# Autodesk Inventor assembly: Intake Full Assembly
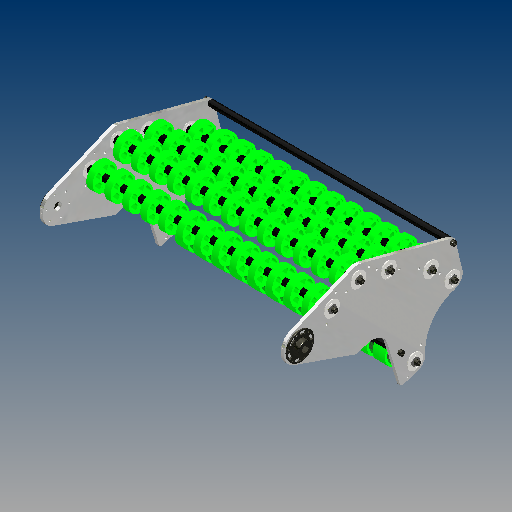
[picture p0: Inventor's stored thumbnail of the model, 512x512]
Saved by Autodesk Inventor 2024.3 (Build 283343000, 343)
## iProperties
Created: 2024-07-29
Part Number: Intake Full Assembly
Document SubType Name: Assembly
Designer: Kenji
Author: Kenji
## Documents named in this file (10)
- C:\Users\Kenji\Documents\GitHub\1622-2024-Summer-CAD-A-Thon\Intake\Intake Full Assembly.iam
- C:\Users\Kenji\Documents\GitHub\1622-2024-Summer-CAD-A-Thon\Intake\Intake Roller Plate.ipt
- C:\Users\Kenji\Documents\GitHub\1622-2024-Summer-CAD-A-Thon\COTS Library\Motion\Bearings\COTS_WCP-0783_1.125ODHexBearing.ipt
- C:\Users\Kenji\Documents\GitHub\1622-2024-Summer-CAD-A-Thon\Intake\Intake HexShaft 1.ipt
- C:\Users\Kenji\Documents\GitHub\1622-2024-Summer-CAD-A-Thon\COTS Library\Motion\Wheels\Compliant Wheels\2in compliant wheels\0.500in hex bore\COTS_am-3462_2indiameter_0.500inhexbore_durometer35A_CompliantWheel.ipt
- C:\Users\Kenji\Documents\GitHub\1622-2024-Summer-CAD-A-Thon\COTS Library\Motion\Wheels\Stealth Wheels\COTS_am-3155 2IN 500Hex Stealth Wheel.iam
- C:\Users\Kenji\Documents\GitHub\1622-2024-Summer-CAD-A-Thon\COTS Library\Structural Adapter\VersaHubs\COTS_217-2592_VersaHub.ipt
- C:\Users\Kenji\Documents\GitHub\1622-2024-Summer-CAD-A-Thon\Intake\Intake BeaterBar.ipt
- C:\Users\Kenji\Documents\GitHub\1622-2024-Summer-CAD-A-Thon\COTS Library\Fasteners\Bolts\Socket-Head\0.25-20\COTS_91251A539_Black-Oxide Alloy Steel Socket Head Screw (1).ipt
- C:\Users\Kenji\Documents\GitHub\1622-2024-Summer-CAD-A-Thon\COTS Library\Fasteners\Washers\COTS_90107A029_316 Stainless Steel Washer.ipt
## Components (129 placed, 9 different names)
1. Intake Roller Plate:1 — Mate:225, Mate:226, Mate:227, Mate:228, Mate:234, Mate:235, Mate:240, Mate:241, Mate:242, Mate:243, Mate:244, Mate:245, Mate:246, Mate:254, Mate:255, Mate:256, Mate:257
2. Intake Roller Plate:2 — Mate:226, Mate:227, Mate:229, Mate:230, Mate:231, Mate:232, Mate:236, Mate:237, Mate:238, Mate:239, Mate:247, Mate:248, Mate:249, Mate:250, Mate:252, Mate:258, Mate:259, Mate:260, Mate:261
3. COTS_WCP-0783_1.125ODHexBearing:1 — Mate:25, Mate:32, Flush:11, Mate:229, Mate:230
4. COTS_WCP-0783_1.125ODHexBearing:2 — Mate:26, Mate:27, Flush:1
5. COTS_WCP-0783_1.125ODHexBearing:3 — Mate:31, Flush:9, Mate:236, Mate:237
6. COTS_WCP-0783_1.125ODHexBearing:4 — Flush:8, Mate:231, Mate:232, Mate:233
7. COTS_WCP-0783_1.125ODHexBearing:5 — Flush:4, Mate:238, Mate:239
8. COTS_WCP-0783_1.125ODHexBearing:6 — Flush:6, Mate:261
9. COTS_WCP-0783_1.125ODHexBearing:7 — Flush:10, Mate:115, Mate:135
10. COTS_WCP-0783_1.125ODHexBearing:8 — Mate:30, Flush:7, Mate:130
11. COTS_WCP-0783_1.125ODHexBearing:9 — Mate:29, Flush:5, Mate:134, Mate:234, Mate:235
12. COTS_WCP-0783_1.125ODHexBearing:10 — Mate:25, Flush:12, Mate:136, Mate:225, Mate:228
13. COTS_WCP-0783_1.125ODHexBearing:11 — Mate:26, Flush:2, Mate:132, Mate:144, Mate:241, Mate:242
14. COTS_WCP-0783_1.125ODHexBearing:12 — Mate:28, Flush:3, Mate:33, Mate:133, Mate:240
15. Intake HexShaft 1:1 — Mate:31, Flush:9, Flush:10, Mate:85, Mate:115, Mate:177, Mate:178, Mate:206, Mate:223
16. Intake HexShaft 1:2 — Mate:32, Flush:11, Flush:12, Mate:98, Mate:183, Mate:184, Mate:209, Mate:220
17. Intake HexShaft 1:3 — Mate:30, Flush:7, Flush:8, Mate:72, Mate:181, Mate:182, Mate:208, Mate:221
18. Intake HexShaft 1:4 — Mate:29, Flush:5, Flush:6, Mate:59, Mate:179, Mate:180, Mate:207, Mate:222
19. Intake HexShaft 1:5 — Mate:28, Flush:3, Flush:4, Mate:175, Mate:176, Mate:205, Mate:224
20. Intake HexShaft 1:6 — Mate:27, Flush:1, Flush:2, Mate:173, Mate:174, Mate:201, Mate:202, Mate:203
21. COTS_217-2592_VersaHub:2 — Mate:255, Mate:256, Mate:257
22. COTS_217-2592_VersaHub:3 — Mate:258, Mate:259, Mate:260
23. Intake BeaterBar:1 — Mate:251, Mate:252
24. Intake BeaterBar:2 — Mate:253, Mate:254
25. COTS_91251A539_Black-Oxide Alloy Steel Socket Head Screw (1):1 — Mate:212, Mate:213
26. COTS_91251A539_Black-Oxide Alloy Steel Socket Head Screw (1):2 — Mate:243, Mate:244, Mate:253
27. COTS_91251A539_Black-Oxide Alloy Steel Socket Head Screw (1):3 — Mate:214, Mate:215
28. COTS_91251A539_Black-Oxide Alloy Steel Socket Head Screw (1):4 — Mate:201, Mate:204
29. COTS_91251A539_Black-Oxide Alloy Steel Socket Head Screw (1):5 — Mate:195, Mate:196
30. COTS_91251A539_Black-Oxide Alloy Steel Socket Head Screw (1):6 — Mate:210, Mate:211
31. COTS_91251A539_Black-Oxide Alloy Steel Socket Head Screw (1):7 — Mate:189, Mate:190
32. COTS_91251A539_Black-Oxide Alloy Steel Socket Head Screw (1):8 — Mate:193, Mate:194
33. COTS_91251A539_Black-Oxide Alloy Steel Socket Head Screw (1):9 — Mate:249, Mate:250, Mate:251
34. COTS_91251A539_Black-Oxide Alloy Steel Socket Head Screw (1):10 — Mate:247, Mate:248
35. COTS_91251A539_Black-Oxide Alloy Steel Socket Head Screw (1):11 — Mate:216, Mate:217
36. COTS_91251A539_Black-Oxide Alloy Steel Socket Head Screw (1):12 — Mate:218, Mate:219
37. COTS_91251A539_Black-Oxide Alloy Steel Socket Head Screw (1):13 — Mate:245, Mate:246
38. COTS_91251A539_Black-Oxide Alloy Steel Socket Head Screw (1):14 — Mate:191, Mate:192
39. COTS_91251A539_Black-Oxide Alloy Steel Socket Head Screw (1):15 — Mate:187, Mate:188, Mate:233
40. COTS_91251A539_Black-Oxide Alloy Steel Socket Head Screw (1):16 — Mate:185, Mate:186
41. COTS_90107A029_316 Stainless Steel Washer:1 — Mate:206, Mate:212, Mate:213, Mate:223
42. COTS_90107A029_316 Stainless Steel Washer:2 — Mate:207, Mate:214, Mate:215, Mate:222
43. COTS_90107A029_316 Stainless Steel Washer:3 — Mate:175, Mate:176, Mate:193, Mate:194
44. COTS_90107A029_316 Stainless Steel Washer:4 — Mate:208, Mate:216, Mate:217, Mate:221
45. COTS_90107A029_316 Stainless Steel Washer:5 — Mate:181, Mate:182, Mate:187, Mate:188
46. COTS_90107A029_316 Stainless Steel Washer:6 — Mate:205, Mate:210, Mate:211, Mate:224
47. COTS_90107A029_316 Stainless Steel Washer:7 — Mate:202, Mate:203, Mate:204
48. COTS_90107A029_316 Stainless Steel Washer:8 — Mate:183, Mate:184, Mate:185, Mate:186
49. COTS_90107A029_316 Stainless Steel Washer:9 — Mate:209, Mate:218, Mate:219, Mate:220
50. COTS_90107A029_316 Stainless Steel Washer:10 — Mate:179, Mate:180, Mate:189, Mate:190
51. COTS_90107A029_316 Stainless Steel Washer:11 — Mate:173, Mate:174, Mate:195, Mate:196
52. COTS_90107A029_316 Stainless Steel Washer:12 — Mate:177, Mate:178, Mate:191, Mate:192
53. COTS_am-3462_2indiameter_0.500inhexbore_durometer35A_CompliantWheel:40 — Mate:72, Mate:130
54. COTS_am-3462_2indiameter_0.500inhexbore_durometer35A_CompliantWheel:53 — Mate:85, Mate:135
55. COTS_am-3462_2indiameter_0.500inhexbore_durometer35A_CompliantWheel:25 — Mate:59, Mate:134
56. COTS_am-3462_2indiameter_0.500inhexbore_durometer35A_CompliantWheel:24 — Mate:33, Mate:133
57. COTS_am-3462_2indiameter_0.500inhexbore_durometer35A_CompliantWheel:66 — Mate:98, Mate:136
58. COTS_am-3462_2indiameter_0.500inhexbore_durometer35A_CompliantWheel:67
59. COTS_am-3462_2indiameter_0.500inhexbore_durometer35A_CompliantWheel:68
60. COTS_am-3462_2indiameter_0.500inhexbore_durometer35A_CompliantWheel:69
61. COTS_am-3462_2indiameter_0.500inhexbore_durometer35A_CompliantWheel:70
62. COTS_am-3462_2indiameter_0.500inhexbore_durometer35A_CompliantWheel:95
63. COTS_am-3462_2indiameter_0.500inhexbore_durometer35A_CompliantWheel:71
64. COTS_am-3462_2indiameter_0.500inhexbore_durometer35A_CompliantWheel:72
65. COTS_am-3462_2indiameter_0.500inhexbore_durometer35A_CompliantWheel:73
66. COTS_am-3462_2indiameter_0.500inhexbore_durometer35A_CompliantWheel:74
67. COTS_am-3462_2indiameter_0.500inhexbore_durometer35A_CompliantWheel:96
68. COTS_am-3462_2indiameter_0.500inhexbore_durometer35A_CompliantWheel:75
69. COTS_am-3462_2indiameter_0.500inhexbore_durometer35A_CompliantWheel:76
70. COTS_am-3462_2indiameter_0.500inhexbore_durometer35A_CompliantWheel:77
71. COTS_am-3462_2indiameter_0.500inhexbore_durometer35A_CompliantWheel:78
72. COTS_am-3462_2indiameter_0.500inhexbore_durometer35A_CompliantWheel:97
73. COTS_am-3462_2indiameter_0.500inhexbore_durometer35A_CompliantWheel:79
74. COTS_am-3462_2indiameter_0.500inhexbore_durometer35A_CompliantWheel:80
75. COTS_am-3462_2indiameter_0.500inhexbore_durometer35A_CompliantWheel:81
76. COTS_am-3462_2indiameter_0.500inhexbore_durometer35A_CompliantWheel:82
77. COTS_am-3462_2indiameter_0.500inhexbore_durometer35A_CompliantWheel:98
78. COTS_am-3462_2indiameter_0.500inhexbore_durometer35A_CompliantWheel:83
79. COTS_am-3462_2indiameter_0.500inhexbore_durometer35A_CompliantWheel:84
80. COTS_am-3462_2indiameter_0.500inhexbore_durometer35A_CompliantWheel:85
81. COTS_am-3462_2indiameter_0.500inhexbore_durometer35A_CompliantWheel:86
82. COTS_am-3462_2indiameter_0.500inhexbore_durometer35A_CompliantWheel:99
83. COTS_am-3462_2indiameter_0.500inhexbore_durometer35A_CompliantWheel:87
84. COTS_am-3462_2indiameter_0.500inhexbore_durometer35A_CompliantWheel:88
85. COTS_am-3462_2indiameter_0.500inhexbore_durometer35A_CompliantWheel:89
86. COTS_am-3462_2indiameter_0.500inhexbore_durometer35A_CompliantWheel:90
87. COTS_am-3462_2indiameter_0.500inhexbore_durometer35A_CompliantWheel:100
88. COTS_am-3462_2indiameter_0.500inhexbore_durometer35A_CompliantWheel:91
89. COTS_am-3462_2indiameter_0.500inhexbore_durometer35A_CompliantWheel:92
90. COTS_am-3462_2indiameter_0.500inhexbore_durometer35A_CompliantWheel:93
91. COTS_am-3462_2indiameter_0.500inhexbore_durometer35A_CompliantWheel:94
92. COTS_am-3462_2indiameter_0.500inhexbore_durometer35A_CompliantWheel:101
93. COTS_am-3462_2indiameter_0.500inhexbore_durometer35A_CompliantWheel:102
94. COTS_am-3462_2indiameter_0.500inhexbore_durometer35A_CompliantWheel:103
95. COTS_am-3462_2indiameter_0.500inhexbore_durometer35A_CompliantWheel:104
96. COTS_am-3462_2indiameter_0.500inhexbore_durometer35A_CompliantWheel:105
97. COTS_am-3462_2indiameter_0.500inhexbore_durometer35A_CompliantWheel:106
98. COTS_am-3462_2indiameter_0.500inhexbore_durometer35A_CompliantWheel:107
99. COTS_am-3462_2indiameter_0.500inhexbore_durometer35A_CompliantWheel:108
100. COTS_am-3462_2indiameter_0.500inhexbore_durometer35A_CompliantWheel:109
101. COTS_am-3462_2indiameter_0.500inhexbore_durometer35A_CompliantWheel:110
102. COTS_am-3462_2indiameter_0.500inhexbore_durometer35A_CompliantWheel:111
103. COTS_am-3462_2indiameter_0.500inhexbore_durometer35A_CompliantWheel:112
104. COTS_am-3462_2indiameter_0.500inhexbore_durometer35A_CompliantWheel:113
105. COTS_am-3462_2indiameter_0.500inhexbore_durometer35A_CompliantWheel:114
106. COTS_am-3462_2indiameter_0.500inhexbore_durometer35A_CompliantWheel:115
107. COTS_am-3462_2indiameter_0.500inhexbore_durometer35A_CompliantWheel:116
108. COTS_am-3462_2indiameter_0.500inhexbore_durometer35A_CompliantWheel:117
109. COTS_am-3462_2indiameter_0.500inhexbore_durometer35A_CompliantWheel:118
110. COTS_am-3462_2indiameter_0.500inhexbore_durometer35A_CompliantWheel:119
111. COTS_am-3462_2indiameter_0.500inhexbore_durometer35A_CompliantWheel:120
112. COTS_am-3462_2indiameter_0.500inhexbore_durometer35A_CompliantWheel:121
113. COTS_am-3462_2indiameter_0.500inhexbore_durometer35A_CompliantWheel:122
114. COTS_am-3462_2indiameter_0.500inhexbore_durometer35A_CompliantWheel:123
115. COTS_am-3462_2indiameter_0.500inhexbore_durometer35A_CompliantWheel:124
116. COTS_am-3462_2indiameter_0.500inhexbore_durometer35A_CompliantWheel:125
117. COTS_am-3462_2indiameter_0.500inhexbore_durometer35A_CompliantWheel:126
118. COTS_am-3155 2IN 500Hex Stealth Wheel:7 [sub-assembly] — Mate:132, Mate:144
119. COTS_am-3155 2IN 500Hex Stealth Wheel:8 [sub-assembly]
120. COTS_am-3155 2IN 500Hex Stealth Wheel:9 [sub-assembly]
121. COTS_am-3155 2IN 500Hex Stealth Wheel:10 [sub-assembly]
122. COTS_am-3155 2IN 500Hex Stealth Wheel:11 [sub-assembly]
123. COTS_am-3155 2IN 500Hex Stealth Wheel:12 [sub-assembly]
124. COTS_am-3155 2IN 500Hex Stealth Wheel:13 [sub-assembly]
125. COTS_am-3155 2IN 500Hex Stealth Wheel:14 [sub-assembly]
126. COTS_am-3155 2IN 500Hex Stealth Wheel:15 [sub-assembly]
127. COTS_am-3155 2IN 500Hex Stealth Wheel:16 [sub-assembly]
128. COTS_am-3155 2IN 500Hex Stealth Wheel:17 [sub-assembly]
129. COTS_am-3155 2IN 500Hex Stealth Wheel:18 [sub-assembly]
## Component patterns: (13 elements, first: COTS_am-3462_2indiameter_0.500inhexbore_durometer35A_CompliantWheel:40 + COTS_am-3462_2indiameter_0.500inhexbore_durometer35A_CompliantWheel:53 + COTS_am-3462_2indiameter_0.500inhexbore_durometer35A_CompliantWheel:25 + COTS_am-3462_2indiameter_0.500inhexbore_durometer35A_CompliantWheel:24 + COTS_am-3462_2indiameter_0.500inhexbore_durometer35A_CompliantWheel:66), (12 elements, first: COTS_am-3155 2IN 500Hex Stealth Wheel:7)
## Relationships (118: Mate 106, Flush 12)
- Mate:25: COTS_WCP-0783_1.125ODHexBearing:1 ↔ COTS_WCP-0783_1.125ODHexBearing:10
- Mate:26: COTS_WCP-0783_1.125ODHexBearing:2 ↔ COTS_WCP-0783_1.125ODHexBearing:11
- Mate:27: COTS_WCP-0783_1.125ODHexBearing:2 ↔ Intake HexShaft 1:6
- Flush:1: COTS_WCP-0783_1.125ODHexBearing:2 ↔ Intake HexShaft 1:6
- Flush:2: COTS_WCP-0783_1.125ODHexBearing:11 ↔ Intake HexShaft 1:6
- Mate:28: COTS_WCP-0783_1.125ODHexBearing:12 ↔ Intake HexShaft 1:5
- Flush:3: COTS_WCP-0783_1.125ODHexBearing:12 ↔ Intake HexShaft 1:5
- Flush:4: COTS_WCP-0783_1.125ODHexBearing:5 ↔ Intake HexShaft 1:5
- Mate:29: COTS_WCP-0783_1.125ODHexBearing:9 ↔ Intake HexShaft 1:4
- Flush:5: COTS_WCP-0783_1.125ODHexBearing:9 ↔ Intake HexShaft 1:4
- Flush:6: COTS_WCP-0783_1.125ODHexBearing:6 ↔ Intake HexShaft 1:4
- Mate:30: COTS_WCP-0783_1.125ODHexBearing:8 ↔ Intake HexShaft 1:3
- Flush:7: COTS_WCP-0783_1.125ODHexBearing:8 ↔ Intake HexShaft 1:3
- Flush:8: COTS_WCP-0783_1.125ODHexBearing:4 ↔ Intake HexShaft 1:3
- Mate:31: COTS_WCP-0783_1.125ODHexBearing:3 ↔ Intake HexShaft 1:1
- Flush:9: COTS_WCP-0783_1.125ODHexBearing:3 ↔ Intake HexShaft 1:1
- Flush:10: COTS_WCP-0783_1.125ODHexBearing:7 ↔ Intake HexShaft 1:1
- Mate:32: COTS_WCP-0783_1.125ODHexBearing:1 ↔ Intake HexShaft 1:2
- Flush:11: COTS_WCP-0783_1.125ODHexBearing:1 ↔ Intake HexShaft 1:2
- Flush:12: COTS_WCP-0783_1.125ODHexBearing:10 ↔ Intake HexShaft 1:2
- Mate:33: COTS_WCP-0783_1.125ODHexBearing:12 ↔ COTS_am-3462_2indiameter_0.500inhexbore_durometer35A_CompliantWheel:24
- Mate:59: Intake HexShaft 1:4 ↔ COTS_am-3462_2indiameter_0.500inhexbore_durometer35A_CompliantWheel:25
- Mate:72: Intake HexShaft 1:3 ↔ COTS_am-3462_2indiameter_0.500inhexbore_durometer35A_CompliantWheel:40
- Mate:85: Intake HexShaft 1:1 ↔ COTS_am-3462_2indiameter_0.500inhexbore_durometer35A_CompliantWheel:53
- Mate:98: Intake HexShaft 1:2 ↔ COTS_am-3462_2indiameter_0.500inhexbore_durometer35A_CompliantWheel:66
- Mate:115: COTS_WCP-0783_1.125ODHexBearing:7 ↔ Intake HexShaft 1:1
- Mate:130 (15.24 mm): COTS_WCP-0783_1.125ODHexBearing:8 ↔ COTS_am-3462_2indiameter_0.500inhexbore_durometer35A_CompliantWheel:40
- Mate:132 (27.94 mm): COTS_WCP-0783_1.125ODHexBearing:11 ↔ COTS_am-3155 2IN 500Hex Stealth Wheel:7
- Mate:133 (15.24 mm): COTS_WCP-0783_1.125ODHexBearing:12 ↔ COTS_am-3462_2indiameter_0.500inhexbore_durometer35A_CompliantWheel:24
- Mate:134 (15.24 mm): COTS_WCP-0783_1.125ODHexBearing:9 ↔ COTS_am-3462_2indiameter_0.500inhexbore_durometer35A_CompliantWheel:25
- Mate:135 (15.24 mm): COTS_WCP-0783_1.125ODHexBearing:7 ↔ COTS_am-3462_2indiameter_0.500inhexbore_durometer35A_CompliantWheel:53
- Mate:136 (15.24 mm): COTS_WCP-0783_1.125ODHexBearing:10 ↔ COTS_am-3462_2indiameter_0.500inhexbore_durometer35A_CompliantWheel:66
- Mate:144: COTS_WCP-0783_1.125ODHexBearing:11 ↔ COTS_am-3155 2IN 500Hex Stealth Wheel:7
- Mate:173: Intake HexShaft 1:6 ↔ COTS_90107A029_316 Stainless Steel Washer:11
- Mate:174: Intake HexShaft 1:6 ↔ COTS_90107A029_316 Stainless Steel Washer:11
- Mate:175: Intake HexShaft 1:5 ↔ COTS_90107A029_316 Stainless Steel Washer:3
- Mate:176: Intake HexShaft 1:5 ↔ COTS_90107A029_316 Stainless Steel Washer:3
- Mate:177: Intake HexShaft 1:1 ↔ COTS_90107A029_316 Stainless Steel Washer:12
- Mate:178: Intake HexShaft 1:1 ↔ COTS_90107A029_316 Stainless Steel Washer:12
- Mate:179: Intake HexShaft 1:4 ↔ COTS_90107A029_316 Stainless Steel Washer:10
- Mate:180: Intake HexShaft 1:4 ↔ COTS_90107A029_316 Stainless Steel Washer:10
- Mate:181: Intake HexShaft 1:3 ↔ COTS_90107A029_316 Stainless Steel Washer:5
- Mate:182: Intake HexShaft 1:3 ↔ COTS_90107A029_316 Stainless Steel Washer:5
- Mate:183: Intake HexShaft 1:2 ↔ COTS_90107A029_316 Stainless Steel Washer:8
- Mate:184: Intake HexShaft 1:2 ↔ COTS_90107A029_316 Stainless Steel Washer:8
- Mate:185: COTS_91251A539_Black-Oxide Alloy Steel Socket Head Screw (1):16 ↔ COTS_90107A029_316 Stainless Steel Washer:8
- Mate:186: COTS_91251A539_Black-Oxide Alloy Steel Socket Head Screw (1):16 ↔ COTS_90107A029_316 Stainless Steel Washer:8
- Mate:187: COTS_91251A539_Black-Oxide Alloy Steel Socket Head Screw (1):15 ↔ COTS_90107A029_316 Stainless Steel Washer:5
- Mate:188: COTS_91251A539_Black-Oxide Alloy Steel Socket Head Screw (1):15 ↔ COTS_90107A029_316 Stainless Steel Washer:5
- Mate:189: COTS_91251A539_Black-Oxide Alloy Steel Socket Head Screw (1):7 ↔ COTS_90107A029_316 Stainless Steel Washer:10
- Mate:190: COTS_91251A539_Black-Oxide Alloy Steel Socket Head Screw (1):7 ↔ COTS_90107A029_316 Stainless Steel Washer:10
- Mate:191: COTS_91251A539_Black-Oxide Alloy Steel Socket Head Screw (1):14 ↔ COTS_90107A029_316 Stainless Steel Washer:12
- Mate:192: COTS_91251A539_Black-Oxide Alloy Steel Socket Head Screw (1):14 ↔ COTS_90107A029_316 Stainless Steel Washer:12
- Mate:193: COTS_91251A539_Black-Oxide Alloy Steel Socket Head Screw (1):8 ↔ COTS_90107A029_316 Stainless Steel Washer:3
- Mate:194: COTS_91251A539_Black-Oxide Alloy Steel Socket Head Screw (1):8 ↔ COTS_90107A029_316 Stainless Steel Washer:3
- Mate:195: COTS_91251A539_Black-Oxide Alloy Steel Socket Head Screw (1):5 ↔ COTS_90107A029_316 Stainless Steel Washer:11
- Mate:196: COTS_91251A539_Black-Oxide Alloy Steel Socket Head Screw (1):5 ↔ COTS_90107A029_316 Stainless Steel Washer:11
- Mate:201: Intake HexShaft 1:6 ↔ COTS_91251A539_Black-Oxide Alloy Steel Socket Head Screw (1):4
- Mate:202: Intake HexShaft 1:6 ↔ COTS_90107A029_316 Stainless Steel Washer:7
- Mate:203: Intake HexShaft 1:6 ↔ COTS_90107A029_316 Stainless Steel Washer:7
- Mate:204: COTS_91251A539_Black-Oxide Alloy Steel Socket Head Screw (1):4 ↔ COTS_90107A029_316 Stainless Steel Washer:7
- Mate:205: Intake HexShaft 1:5 ↔ COTS_90107A029_316 Stainless Steel Washer:6
- Mate:206: Intake HexShaft 1:1 ↔ COTS_90107A029_316 Stainless Steel Washer:1
- Mate:207: Intake HexShaft 1:4 ↔ COTS_90107A029_316 Stainless Steel Washer:2
- Mate:208: Intake HexShaft 1:3 ↔ COTS_90107A029_316 Stainless Steel Washer:4
- Mate:209: Intake HexShaft 1:2 ↔ COTS_90107A029_316 Stainless Steel Washer:9
- Mate:210: COTS_91251A539_Black-Oxide Alloy Steel Socket Head Screw (1):6 ↔ COTS_90107A029_316 Stainless Steel Washer:6
- Mate:211: COTS_91251A539_Black-Oxide Alloy Steel Socket Head Screw (1):6 ↔ COTS_90107A029_316 Stainless Steel Washer:6
- Mate:212: COTS_91251A539_Black-Oxide Alloy Steel Socket Head Screw (1):1 ↔ COTS_90107A029_316 Stainless Steel Washer:1
- Mate:213: COTS_91251A539_Black-Oxide Alloy Steel Socket Head Screw (1):1 ↔ COTS_90107A029_316 Stainless Steel Washer:1
- Mate:214: COTS_91251A539_Black-Oxide Alloy Steel Socket Head Screw (1):3 ↔ COTS_90107A029_316 Stainless Steel Washer:2
- Mate:215: COTS_91251A539_Black-Oxide Alloy Steel Socket Head Screw (1):3 ↔ COTS_90107A029_316 Stainless Steel Washer:2
- Mate:216: COTS_91251A539_Black-Oxide Alloy Steel Socket Head Screw (1):11 ↔ COTS_90107A029_316 Stainless Steel Washer:4
- Mate:217: COTS_91251A539_Black-Oxide Alloy Steel Socket Head Screw (1):11 ↔ COTS_90107A029_316 Stainless Steel Washer:4
- Mate:218: COTS_91251A539_Black-Oxide Alloy Steel Socket Head Screw (1):12 ↔ COTS_90107A029_316 Stainless Steel Washer:9
- Mate:219: COTS_91251A539_Black-Oxide Alloy Steel Socket Head Screw (1):12 ↔ COTS_90107A029_316 Stainless Steel Washer:9
- Mate:220: Intake HexShaft 1:2 ↔ COTS_90107A029_316 Stainless Steel Washer:9
- Mate:221: Intake HexShaft 1:3 ↔ COTS_90107A029_316 Stainless Steel Washer:4
- Mate:222: Intake HexShaft 1:4 ↔ COTS_90107A029_316 Stainless Steel Washer:2
- Mate:223: Intake HexShaft 1:1 ↔ COTS_90107A029_316 Stainless Steel Washer:1
- Mate:224: Intake HexShaft 1:5 ↔ COTS_90107A029_316 Stainless Steel Washer:6
- Mate:225: Intake Roller Plate:1 ↔ COTS_WCP-0783_1.125ODHexBearing:10
- Mate:226: Intake Roller Plate:1 ↔ Intake Roller Plate:2
- Mate:227: Intake Roller Plate:1 ↔ Intake Roller Plate:2
- Mate:228: Intake Roller Plate:1 ↔ COTS_WCP-0783_1.125ODHexBearing:10
- Mate:229: Intake Roller Plate:2 ↔ COTS_WCP-0783_1.125ODHexBearing:1
- Mate:230: Intake Roller Plate:2 ↔ COTS_WCP-0783_1.125ODHexBearing:1
- Mate:231: Intake Roller Plate:2 ↔ COTS_WCP-0783_1.125ODHexBearing:4
- Mate:232: Intake Roller Plate:2 ↔ COTS_WCP-0783_1.125ODHexBearing:4
- Mate:233: COTS_WCP-0783_1.125ODHexBearing:4 ↔ COTS_91251A539_Black-Oxide Alloy Steel Socket Head Screw (1):15
- Mate:234: Intake Roller Plate:1 ↔ COTS_WCP-0783_1.125ODHexBearing:9
- Mate:235: Intake Roller Plate:1 ↔ COTS_WCP-0783_1.125ODHexBearing:9
- Mate:236: Intake Roller Plate:2 ↔ COTS_WCP-0783_1.125ODHexBearing:3
- Mate:237: Intake Roller Plate:2 ↔ COTS_WCP-0783_1.125ODHexBearing:3
- Mate:238: Intake Roller Plate:2 ↔ COTS_WCP-0783_1.125ODHexBearing:5
- Mate:239: Intake Roller Plate:2 ↔ COTS_WCP-0783_1.125ODHexBearing:5
- Mate:240: Intake Roller Plate:1 ↔ COTS_WCP-0783_1.125ODHexBearing:12
- Mate:241: Intake Roller Plate:1 ↔ COTS_WCP-0783_1.125ODHexBearing:11
- Mate:242: Intake Roller Plate:1 ↔ COTS_WCP-0783_1.125ODHexBearing:11
- Mate:243: Intake Roller Plate:1 ↔ COTS_91251A539_Black-Oxide Alloy Steel Socket Head Screw (1):2
- Mate:244: Intake Roller Plate:1 ↔ COTS_91251A539_Black-Oxide Alloy Steel Socket Head Screw (1):2
- Mate:245: Intake Roller Plate:1 ↔ COTS_91251A539_Black-Oxide Alloy Steel Socket Head Screw (1):13
- Mate:246: Intake Roller Plate:1 ↔ COTS_91251A539_Black-Oxide Alloy Steel Socket Head Screw (1):13
- Mate:247: Intake Roller Plate:2 ↔ COTS_91251A539_Black-Oxide Alloy Steel Socket Head Screw (1):10
- Mate:248: Intake Roller Plate:2 ↔ COTS_91251A539_Black-Oxide Alloy Steel Socket Head Screw (1):10
- Mate:249: Intake Roller Plate:2 ↔ COTS_91251A539_Black-Oxide Alloy Steel Socket Head Screw (1):9
- Mate:250: Intake Roller Plate:2 ↔ COTS_91251A539_Black-Oxide Alloy Steel Socket Head Screw (1):9
- Mate:251: Intake BeaterBar:1 ↔ COTS_91251A539_Black-Oxide Alloy Steel Socket Head Screw (1):9
- Mate:252: Intake Roller Plate:2 ↔ Intake BeaterBar:1
- Mate:253: Intake BeaterBar:2 ↔ COTS_91251A539_Black-Oxide Alloy Steel Socket Head Screw (1):2
- Mate:254: Intake Roller Plate:1 ↔ Intake BeaterBar:2
- Mate:255: Intake Roller Plate:1 ↔ COTS_217-2592_VersaHub:2
- Mate:256: Intake Roller Plate:1 ↔ COTS_217-2592_VersaHub:2
- Mate:257: Intake Roller Plate:1 ↔ COTS_217-2592_VersaHub:2
- Mate:258: Intake Roller Plate:2 ↔ COTS_217-2592_VersaHub:3
- Mate:259: Intake Roller Plate:2 ↔ COTS_217-2592_VersaHub:3
- Mate:260: Intake Roller Plate:2 ↔ COTS_217-2592_VersaHub:3
- Mate:261: Intake Roller Plate:2 ↔ COTS_WCP-0783_1.125ODHexBearing:6
